# Autodesk Inventor assembly: Big Bearing Cover Assembled
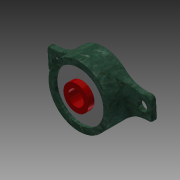
[picture p0: Inventor's stored thumbnail of the model, 180x180]
Saved by Autodesk Inventor 2014 (Build 180170000, 170)
## iProperties
Created: 2015-02-12
Part Number: Big Bearing Cover Assembled
Document SubType Name: Assembly
Designer: Spooner
Author: Spooner
## Documents named in this file (4)
- C:\Users\Spooner\Documents\Inventor\80-20  Linear Bearing\Big Bearing Cover Assembled.iam
- C:\Users\Spooner\Documents\Inventor\80-20  Linear Bearing\Big Bearing.ipt
- C:\Users\Spooner\Documents\Inventor\80-20  Linear Bearing\Big Bearing Sleeve.ipt
- C:\Users\Spooner\Documents\Inventor\80-20  Linear Bearing\Big Bearing Mount.ipt
## Components (3 placed, 3 different names)
1. Big Bearing:1 — Insert:1, Insert:2
2. Big Bearing Sleeve:1 — Insert:2
3. Big Bearing Mount:1 — Insert:1
## Relationships (2: Insert 2)
- Insert:1: Big Bearing:1 ↔ Big Bearing Mount:1
- Insert:2: Big Bearing:1 ↔ Big Bearing Sleeve:1
